# Autodesk Inventor assembly: wheel assemblyMirrored
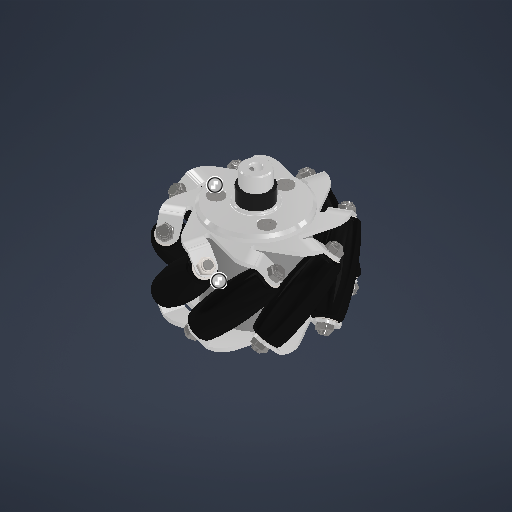
[picture p0: Inventor's stored thumbnail of the model, 512x512]
Saved by Autodesk Inventor 2025 (Build 290162000, 162)
## iProperties
Created: 2023-06-24
Part Number: wheel assemblyMirrored
Document SubType Name: Assembly
Designer: khrip
Mass: 107.295 g
Surface Area: 386.365 cm^2
Volume: 54.6178 cm^3
Density: 1.96447 g/cm^3
Author: khrip
## Documents named in this file (9)
- H:\Botik\Chassis\UnsprungUnits\Wheels\wheel assemblyMirrored.iam
- H:\Botik\Chassis\UnsprungUnits\Wheels\wheelAss\Mecanum_Wheel_60mm_Right_ASM_AP214Mirrored.iam
- H:\Botik\Chassis\UnsprungUnits\Wheels\Parts\fittingRingInstalled.ipt
- H:\Botik\Chassis\UnsprungUnits\Wheels\Parts\washer.ipt
- H:\Botik\Chassis\UnsprungUnits\Wheels\Parts\wheelHub.ipt
- C:\Users\khrip\Documents\Inventor\Content Center Files\R2025\ru-RU\GOST 17475-80 (2)\Винт 2.M3-6gx40 ГОСТ 17475-80.ipt
- C:\Users\khrip\Documents\Inventor\Content Center Files\R2025\ru-RU\DIN 985\DIN 985 - M3.ipt
- C:\Users\khrip\Documents\Inventor\Content Center Files\R2025\ru-RU\GOST 9649-78\Шайба 3 ГОСТ 9649-78.ipt
- C:\Users\khrip\Documents\Inventor\Content Center Files\R2025\ru-RU\GOST 17475-80 (2)\Винт 2.M4-6gx40 ГОСТ 17475-80.ipt
## Components (14 placed, 8 different names)
1. Mecanum_Wheel_60mm_Right_ASM_AP214Mirrored:1 [sub-assembly] — Совмещение:3, Совмещение:4, Совмещение:5, Совмещение:6, Совмещение:7, Совмещение:8, Совмещение:20, Совмещение:22, Совмещение:24
2. fittingRingInstalled:1 — Совмещение:9, Совмещение:10
3. washer:1 — Совмещение:6, Совмещение:7, Совмещение:8, Совмещение:25
4. wheelHub:1 — Совмещение:1, Угол:1, Совмещение:2, Совмещение:3, Совмещение:4, Совмещение:5, Совмещение:9, Совмещение:10, Совмещение:16, Совмещение:17, Совмещение:18, Совмещение:19, Совмещение:21, Совмещение:23
5. Винт 2 ГОСТ 17475-80 M3 x 40:1 — Совмещение:16
6. DIN 985 - заменено на DIN EN ISO 10511 M3:1 — Вставка:1
7. Шайба ГОСТ 9649-78 3:1 — Совмещение:19, Совмещение:20, Вставка:1
8. Винт 2 ГОСТ 17475-80 M3 x 40:2 — Совмещение:17
9. Винт 2 ГОСТ 17475-80 M3 x 40:3 — Совмещение:18
10. Шайба ГОСТ 9649-78 3:2 — Совмещение:21, Совмещение:22, Вставка:2
11. Шайба ГОСТ 9649-78 3:3 — Совмещение:23, Совмещение:24, Вставка:3
12. DIN 985 - заменено на DIN EN ISO 10511 M3:2 — Вставка:2
13. DIN 985 - заменено на DIN EN ISO 10511 M3:3 — Вставка:3
14. Винт 2 ГОСТ 17475-80 M4 x 40:1 — Совмещение:25
## Relationships (24: Mate 20, Insert 3, Angle 1)
- Совмещение:1 [Mate] (16 mm): wheelHub:1
- Угол:1 [Angle] (0 deg): wheelHub:1
- Совмещение:2 [Mate]: wheelHub:1
- Совмещение:3 [Mate]: Mecanum_Wheel_60mm_Right_ASM_AP214Mirrored:1 ↔ wheelHub:1
- Совмещение:4 [Mate]: Mecanum_Wheel_60mm_Right_ASM_AP214Mirrored:1 ↔ wheelHub:1
- Совмещение:5 [Mate]: Mecanum_Wheel_60mm_Right_ASM_AP214Mirrored:1 ↔ wheelHub:1
- Совмещение:6 [Mate]: Mecanum_Wheel_60mm_Right_ASM_AP214Mirrored:1 ↔ washer:1
- Совмещение:7 [Mate]: Mecanum_Wheel_60mm_Right_ASM_AP214Mirrored:1 ↔ washer:1
- Совмещение:8 [Mate]: Mecanum_Wheel_60mm_Right_ASM_AP214Mirrored:1 ↔ washer:1
- Совмещение:9 [Mate]: fittingRingInstalled:1 ↔ wheelHub:1
- Совмещение:10 [Mate]: fittingRingInstalled:1 ↔ wheelHub:1
- Совмещение:16 [Mate]: wheelHub:1 ↔ Винт 2 ГОСТ 17475-80 M3 x 40:1
- Совмещение:17 [Mate]: wheelHub:1 ↔ Винт 2 ГОСТ 17475-80 M3 x 40:2
- Совмещение:18 [Mate]: wheelHub:1 ↔ Винт 2 ГОСТ 17475-80 M3 x 40:3
- Совмещение:19 [Mate]: wheelHub:1 ↔ Шайба ГОСТ 9649-78 3:1
- Совмещение:20 [Mate]: Mecanum_Wheel_60mm_Right_ASM_AP214Mirrored:1 ↔ Шайба ГОСТ 9649-78 3:1
- Совмещение:21 [Mate]: wheelHub:1 ↔ Шайба ГОСТ 9649-78 3:2
- Совмещение:22 [Mate]: Mecanum_Wheel_60mm_Right_ASM_AP214Mirrored:1 ↔ Шайба ГОСТ 9649-78 3:2
- Совмещение:23 [Mate]: wheelHub:1 ↔ Шайба ГОСТ 9649-78 3:3
- Совмещение:24 [Mate]: Mecanum_Wheel_60mm_Right_ASM_AP214Mirrored:1 ↔ Шайба ГОСТ 9649-78 3:3
- Вставка:1 [Insert]: DIN 985 - заменено на DIN EN ISO 10511 M3:1 ↔ Шайба ГОСТ 9649-78 3:1
- Вставка:2 [Insert]: Шайба ГОСТ 9649-78 3:2 ↔ DIN 985 - заменено на DIN EN ISO 10511 M3:2
- Вставка:3 [Insert]: Шайба ГОСТ 9649-78 3:3 ↔ DIN 985 - заменено на DIN EN ISO 10511 M3:3
- Совмещение:25 [Mate]: washer:1 ↔ Винт 2 ГОСТ 17475-80 M4 x 40:1
